# Autodesk Inventor assembly: 3D_PCB4_2024-01-15
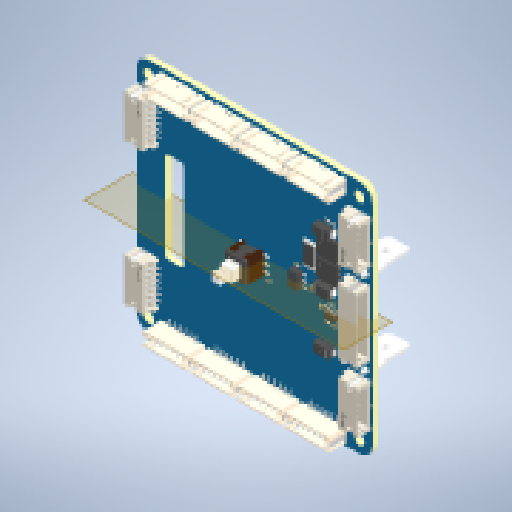
[picture p0: Inventor's stored thumbnail of the model, 512x512]
Saved by Autodesk Inventor 2024.2 (Build 282272000, 272)
## iProperties
Created: 2025-09-19
Part Number: 3D_PCB4_2024-01-15
Document SubType Name: Assembly
Designer: AdminForWorker
Title: 3D_PCB4_2024-01-15 v3
Author: AdminForWorker
## Documents named in this file (38)
- C:\dog\Pupper+v3\3D_PCB4_2024-01-15 v3.iam
- C:\dog\Pupper+v3\Board.ipt
- C:\dog\Pupper+v3\Q2.iam
- C:\dog\Pupper+v3\Q1.iam
- C:\dog\Pupper+v3\SW1.iam
- C:\dog\Pupper+v3\R15.iam
- C:\dog\Pupper+v3\J2.iam
- C:\dog\Pupper+v3\J1.iam
- C:\dog\Pupper+v3\U40.iam
- C:\dog\Pupper+v3\U42.iam
- C:\dog\Pupper+v3\D3.iam
- C:\dog\Pupper+v3\D2.iam
- C:\dog\Pupper+v3\R16.iam
- C:\dog\Pupper+v3\R12.iam
- C:\dog\Pupper+v3\R8.iam
- C:\dog\Pupper+v3\R9.iam
- C:\dog\Pupper+v3\R11.iam
- C:\dog\Pupper+v3\R14.iam
- C:\dog\Pupper+v3\R17.iam
- C:\dog\Pupper+v3\R22.iam
- C:\dog\Pupper+v3\R7.iam
- C:\dog\Pupper+v3\CN17.iam
- C:\dog\Pupper+v3\CN7.iam
- C:\dog\Pupper+v3\CN9.iam
- C:\dog\Pupper+v3\CN10.iam
- C:\dog\Pupper+v3\CN12.iam
- C:\dog\Pupper+v3\CN13.iam
- C:\dog\Pupper+v3\CN15.iam
- C:\dog\Pupper+v3\CN16.iam
- C:\dog\Pupper+v3\CN6.iam
- C:\dog\Pupper+v3\C50.iam
- C:\dog\Pupper+v3\C52.iam
- C:\dog\Pupper+v3\C51.iam
- C:\dog\Pupper+v3\D4.iam
- C:\dog\Pupper+v3\CN8.iam
- C:\dog\Pupper+v3\CN11.iam
- C:\dog\Pupper+v3\CN14.iam
- C:\dog\Pupper+v3\CN5.iam
## Components (37 placed, 37 different names)
1. Board:1 — Угол:1
2. Q2:1 [sub-assembly]
3. Q1:1 [sub-assembly]
4. SW1:1 [sub-assembly] — Совмещение:1
5. R15:1 [sub-assembly]
6. J2:1 [sub-assembly]
7. J1:1 [sub-assembly]
8. U40:1 [sub-assembly]
9. U42:1 [sub-assembly]
10. D3:1 [sub-assembly]
11. D2:1 [sub-assembly]
12. R16:1 [sub-assembly]
13. R12:1 [sub-assembly]
14. R8:1 [sub-assembly]
15. R9:1 [sub-assembly]
16. R11:1 [sub-assembly]
17. R14:1 [sub-assembly]
18. R17:1 [sub-assembly]
19. R22:1 [sub-assembly]
20. R7:1 [sub-assembly]
21. CN17:1 [sub-assembly]
22. CN7:1 [sub-assembly]
23. CN9:1 [sub-assembly]
24. CN10:1 [sub-assembly]
25. CN12:1 [sub-assembly]
26. CN13:1 [sub-assembly]
27. CN15:1 [sub-assembly]
28. CN16:1 [sub-assembly]
29. CN6:1 [sub-assembly]
30. C50:1 [sub-assembly]
31. C52:1 [sub-assembly]
32. C51:1 [sub-assembly]
33. D4:1 [sub-assembly]
34. CN8:1 [sub-assembly]
35. CN11:1 [sub-assembly]
36. CN14:1 [sub-assembly]
37. CN5:1 [sub-assembly]
## Relationships (2: Mate 1, Angle 1)
- Совмещение:1 [Mate]: SW1:1
- Угол:1 [Angle] (0 deg): Board:1
